# Autodesk Inventor assembly: FullArmAJB
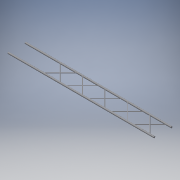
[picture p0: Inventor's stored thumbnail of the model, 180x180]
Saved by Autodesk Inventor 2018 (Build 220112000, 112)
## iProperties
Created: 2018-02-16
Part Number: FullArmAJB
Document SubType Name: Assembly
Designer: Alec temporary
Author: Alec temporary
## Documents named in this file (3)
- M:\TPS\9th Grade\CADD 2017-2018\Current\Ferris Wheel Group Project\Group Project Week 3\FullArmAJB.iam
- M:\TPS\9th Grade\CADD 2017-2018\Current\Ferris Wheel Group Project\Group Project Week 3\FullRadiusPoleAJB.iam
- M:\TPS\9th Grade\CADD 2017-2018\Current\Ferris Wheel Group Project\Group Project Week 3\CrossbeamPoleAJB.ipt
## Components (7 placed, 2 different names)
1. FullRadiusPoleAJB:1 [sub-assembly] — Flush:1, Mate:1, Flush:2, Flush:3, Mate:3, Flush:6, Mate:4, Mate:7, Mate:8, Mate:9, Mate:10, Mate:11, Mate:12, Mate:13, Mate:14, Mate:15, Mate:16
2. FullRadiusPoleAJB:2 [sub-assembly] — Flush:1, Mate:1, Flush:2, Mate:5, Mate:6, Flush:7, Symmetry:1
3. CrossbeamPoleAJB:1 — Flush:3, Flush:4, Flush:5
4. CrossbeamPoleAJB:2 — Mate:5, Mate:6, Mate:7
5. CrossbeamPoleAJB:3 — Mate:8, Mate:9, Mate:10
6. CrossbeamPoleAJB:4 — Mate:11, Mate:12, Mate:13
7. CrossbeamPoleAJB:5 — Mate:14, Mate:15, Mate:16
## Relationships (26: Mate 18, Flush 7, Symmetry 1)
- Flush:1: FullRadiusPoleAJB:1 ↔ FullRadiusPoleAJB:2
- Mate:1: FullRadiusPoleAJB:1 ↔ FullRadiusPoleAJB:2
- Flush:2 (-2692.4 mm): FullRadiusPoleAJB:1 ↔ FullRadiusPoleAJB:2
- Flush:3: FullRadiusPoleAJB:1 ↔ CrossbeamPoleAJB:1
- Flush:4: CrossbeamPoleAJB:1
- Flush:5: CrossbeamPoleAJB:1
- Mate:2
- Mate:3: FullRadiusPoleAJB:1
- Flush:6: FullRadiusPoleAJB:1
- Mate:4: FullRadiusPoleAJB:1
- Mate:5: FullRadiusPoleAJB:2 ↔ CrossbeamPoleAJB:2
- Mate:6: FullRadiusPoleAJB:2 ↔ CrossbeamPoleAJB:2
- Mate:7: FullRadiusPoleAJB:1 ↔ CrossbeamPoleAJB:2
- Mate:8: FullRadiusPoleAJB:1 ↔ CrossbeamPoleAJB:3
- Mate:9: FullRadiusPoleAJB:1 ↔ CrossbeamPoleAJB:3
- Mate:10: FullRadiusPoleAJB:1 ↔ CrossbeamPoleAJB:3
- Mate:11: FullRadiusPoleAJB:1 ↔ CrossbeamPoleAJB:4
- Mate:12: FullRadiusPoleAJB:1 ↔ CrossbeamPoleAJB:4
- Mate:13: FullRadiusPoleAJB:1 ↔ CrossbeamPoleAJB:4
- Mate:14: FullRadiusPoleAJB:1 ↔ CrossbeamPoleAJB:5
- Mate:15: FullRadiusPoleAJB:1 ↔ CrossbeamPoleAJB:5
- Mate:16: FullRadiusPoleAJB:1 ↔ CrossbeamPoleAJB:5
- Flush:7: FullRadiusPoleAJB:2
- Symmetry:1: FullRadiusPoleAJB:2
- Mate:17
- Mate:18
